# Autodesk Inventor assembly: vdpillar_printasm
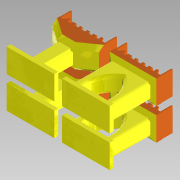
[picture p0: Inventor's stored thumbnail of the model, 180x180]
Saved by Autodesk Inventor 2021 (Build 250183000, 183)
## iProperties
Created: 2021-03-10
Part Number: vdpillar_printasm
Document SubType Name: Assembly
Designer: kumagai
Author: kumagai
## Documents named in this file (3)
- X:\Develop\CAD\PlaRails\ViaductPillar\vdpillar_printasm.iam
- X:\Develop\CAD\PlaRails\ViaductPillar\VDPillar_A_C.ipt
- X:\Develop\CAD\PlaRails\ViaductPillar\VDPillar_B_C.ipt
## Components (4 placed, 2 different names)
1. VDPillar_A_C:1
2. VDPillar_B_C:1 — フラッシュ:1, フラッシュ:2, フラッシュ:3
3. VDPillar_A_C:2
4. VDPillar_B_C:2
## Component patterns: (2 elements, first: VDPillar_A_C:1 + VDPillar_B_C:1)
## Relationships (3: Flush 3)
- フラッシュ:1 [Flush] (70 mm): VDPillar_B_C:1
- フラッシュ:2 [Flush]: VDPillar_B_C:1
- フラッシュ:3 [Flush]: VDPillar_B_C:1
